# Autodesk Inventor assembly: sorting and interface V2
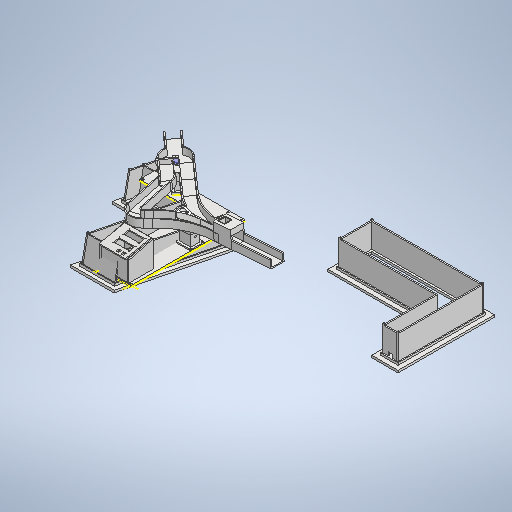
[picture p0: Inventor's stored thumbnail of the model, 512x512]
Saved by Autodesk Inventor 2025.3 (Build 293356000, 356)
## iProperties
Created: 2026-04-18
Part Number: sorting and interface V2
Document SubType Name: Assembly
Designer: kamal
Author: kamal
## Documents named in this file (30)
- C:\Users\kamal\OneDrive\Desktop\Personal\semester 4\Basics of Mechatronics\Full Assembly\sorting and interface V2.iam
- C:\Users\kamal\OneDrive\Desktop\Personal\semester 4\Basics of Mechatronics\Full Assembly\Sorting Full Mechanism.iam
- C:\Users\kamal\OneDrive\Desktop\Personal\semester 4\Basics of Mechatronics\Full Assembly\track 1832.ipt
- C:\Users\kamal\OneDrive\Desktop\Personal\semester 4\Basics of Mechatronics\Full Assembly\track z1906.ipt
- C:\Users\kamal\OneDrive\Desktop\Personal\semester 4\Basics of Mechatronics\Full Assembly\selection system 2.iam
- C:\Users\kamal\OneDrive\Desktop\Personal\semester 4\Basics of Mechatronics\Full Assembly\track z2029.ipt
- C:\Users\kamal\OneDrive\Desktop\Personal\semester 4\Basics of Mechatronics\Full Assembly\track z2053.ipt
- C:\Users\kamal\OneDrive\Desktop\Personal\semester 4\Basics of Mechatronics\Full Assembly\track z2059.ipt
- C:\Users\kamal\OneDrive\Desktop\Personal\semester 4\Basics of Mechatronics\Full Assembly\select end track.ipt
- C:\Users\kamal\OneDrive\Desktop\Personal\semester 4\Basics of Mechatronics\Full Assembly\sort support V3.ipt
- C:\Users\kamal\OneDrive\Desktop\Personal\semester 4\Basics of Mechatronics\Full Assembly\select support V3.ipt
- C:\Users\kamal\OneDrive\Desktop\Personal\semester 4\Basics of Mechatronics\Full Assembly\base zzzz.ipt
- C:\Users\kamal\OneDrive\Desktop\Personal\semester 4\Basics of Mechatronics\Full Assembly\wall inteface V1.ipt
- C:\Users\kamal\OneDrive\Desktop\Personal\semester 4\Basics of Mechatronics\Full Assembly\wall interface 2 V1.ipt
- C:\Users\kamal\OneDrive\Desktop\Personal\semester 4\Basics of Mechatronics\Full Assembly\lcd holder.ipt
- C:\Users\kamal\OneDrive\Desktop\Personal\semester 4\Basics of Mechatronics\Full Assembly\wall interface 3 V1.ipt
- C:\Users\kamal\OneDrive\Desktop\Personal\semester 4\Basics of Mechatronics\Full Assembly\base down.ipt
- C:\Users\kamal\OneDrive\Desktop\Personal\semester 4\Basics of Mechatronics\Full Assembly\wall 1 for sorting.ipt
- C:\Users\kamal\OneDrive\Desktop\Personal\semester 4\Basics of Mechatronics\Full Assembly\wall 2 for sorting.ipt
- C:\Users\kamal\OneDrive\Desktop\Personal\semester 4\Basics of Mechatronics\Full Assembly\wall 3 for sorting.ipt
- C:\Users\kamal\OneDrive\Desktop\Personal\semester 4\Basics of Mechatronics\Full Assembly\wall 4 for sorting.ipt
- C:\Users\kamal\OneDrive\Desktop\Personal\semester 4\Basics of Mechatronics\Full Assembly\wall 5 for sorting.ipt
- C:\Users\kamal\OneDrive\Desktop\Personal\semester 4\Basics of Mechatronics\Full Assembly\wall 6 for sorting.ipt
- C:\Users\kamal\OneDrive\Desktop\Personal\semester 4\Basics of Mechatronics\Full Assembly\base down_MIR.ipt
- C:\Users\kamal\OneDrive\Desktop\Personal\semester 4\Basics of Mechatronics\Full Assembly\wall 1 for sorting_MIR.ipt
- C:\Users\kamal\OneDrive\Desktop\Personal\semester 4\Basics of Mechatronics\Full Assembly\wall 2 for sorting_MIR.ipt
- C:\Users\kamal\OneDrive\Desktop\Personal\semester 4\Basics of Mechatronics\Full Assembly\wall 3 for sorting_MIR.ipt
- C:\Users\kamal\OneDrive\Desktop\Personal\semester 4\Basics of Mechatronics\Full Assembly\wall 4 for sorting_MIR.ipt
- C:\Users\kamal\OneDrive\Desktop\Personal\semester 4\Basics of Mechatronics\Full Assembly\wall 5 for sorting_MIR.ipt
- C:\Users\kamal\OneDrive\Desktop\Personal\semester 4\Basics of Mechatronics\Full Assembly\wall 6 for sorting_MIR.ipt
## Components (31 placed, 29 different names)
1. Sorting Full Mechanism:1 [sub-assembly] — Mate:12, Mate:13, Mate:14, Mate:21, Mate:22, Mate:25, Mate:26, Mate:56, Mate:57
2. track 1832:1 — Mate:12, Mate:13, Mate:14
3. track z1906:1 — Mate:21, Mate:22, Mate:52, Mate:53
4. selection system 2:1 [sub-assembly] — Mate:27, Mate:28, Mate:41, Mate:42, Mate:54, Mate:55, Mate:58, Mate:59
5. track z2029:1 — Mate:25, Mate:26, Mate:27, Mate:28
6. track z1906:3 — Mate:35, Mate:36, Mate:52, Mate:53
7. track z2053:1 — Mate:35, Mate:36
8. track z2059:1 — Mate:54, Mate:55
9. select end track:1 — Mate:41, Mate:42
10. sort support V3:1 — Mate:56, Mate:57, Mate:60, Mate:61
11. select support V3:1 — Mate:58, Mate:59
12. base zzzz:1 — Mate:60, Mate:61, Mate:62, Mate:63, Mate:64, Mate:65, Mate:68, Mate:70, Mate:98
13. wall inteface V1:1 — Mate:64, Mate:65, Mate:66, Mate:69, Mate:72
14. wall interface 2 V1:1 — Mate:62, Mate:63, Mate:67, Mate:71
15. lcd holder:1 — Mate:66
16. wall interface 3 V1:1 — Mate:69, Mate:70, Mate:71
17. wall interface 3 V1:2 — Mate:67, Mate:68, Mate:72
18. base down:1 — Mate:73, Mate:74, Mate:75, Mate:76, Mate:77, Mate:78, Mate:79, Mate:80, Mate:81, Mate:82, Mate:84
19. wall 1 for sorting:1 — Mate:73, Mate:74, Mate:85
20. wall 2 for sorting:1 — Mate:75, Mate:76
21. wall 3 for sorting:1 — Mate:77, Mate:78
22. wall 4 for sorting:1 — Mate:79, Mate:80
23. wall 5 for sorting:2 — Mate:81, Mate:82
24. wall 6 for sorting:1 — Mate:84, Mate:85
25. base down_MIR:1 — Mate:86, Mate:87, Mate:88, Mate:89, Mate:90, Mate:91, Mate:92, Mate:93, Mate:94, Mate:95, Mate:97
26. wall 1 for sorting_MIR:1 — Mate:86, Mate:87, Mate:96
27. wall 2 for sorting_MIR:1 — Mate:88, Mate:89, Mate:98
28. wall 3 for sorting_MIR:1 — Mate:90, Mate:91
29. wall 4 for sorting_MIR:1 — Mate:92, Mate:93
30. wall 5 for sorting_MIR:1 — Mate:94, Mate:95
31. wall 6 for sorting_MIR:1 — Mate:96, Mate:97
## Relationships (59: Mate 59)
- Mate:12: Sorting Full Mechanism:1 ↔ track 1832:1
- Mate:13: Sorting Full Mechanism:1 ↔ track 1832:1
- Mate:14: Sorting Full Mechanism:1 ↔ track 1832:1
- Mate:21: Sorting Full Mechanism:1 ↔ track z1906:1
- Mate:22: Sorting Full Mechanism:1 ↔ track z1906:1
- Mate:25: Sorting Full Mechanism:1 ↔ track z2029:1
- Mate:26: Sorting Full Mechanism:1 ↔ track z2029:1
- Mate:27: selection system 2:1 ↔ track z2029:1
- Mate:28: selection system 2:1 ↔ track z2029:1
- Mate:35: track z1906:3 ↔ track z2053:1
- Mate:36: track z1906:3 ↔ track z2053:1
- Mate:41: selection system 2:1 ↔ select end track:1
- Mate:42: selection system 2:1 ↔ select end track:1
- Mate:52: track z1906:1 ↔ track z1906:3
- Mate:53: track z1906:1 ↔ track z1906:3
- Mate:54: selection system 2:1 ↔ track z2059:1
- Mate:55: selection system 2:1 ↔ track z2059:1
- Mate:56: Sorting Full Mechanism:1 ↔ sort support V3:1
- Mate:57: Sorting Full Mechanism:1 ↔ sort support V3:1
- Mate:58: selection system 2:1 ↔ select support V3:1
- Mate:59 (5 mm): selection system 2:1 ↔ select support V3:1
- Mate:60: sort support V3:1 ↔ base zzzz:1
- Mate:61: sort support V3:1 ↔ base zzzz:1
- Mate:62: base zzzz:1 ↔ wall interface 2 V1:1
- Mate:63: base zzzz:1 ↔ wall interface 2 V1:1
- Mate:64: base zzzz:1 ↔ wall inteface V1:1
- Mate:65: base zzzz:1 ↔ wall inteface V1:1
- Mate:66: wall inteface V1:1 ↔ lcd holder:1
- Mate:67: wall interface 2 V1:1 ↔ wall interface 3 V1:2
- Mate:68: base zzzz:1 ↔ wall interface 3 V1:2
- Mate:69: wall inteface V1:1 ↔ wall interface 3 V1:1
- Mate:70: base zzzz:1 ↔ wall interface 3 V1:1
- Mate:71: wall interface 2 V1:1 ↔ wall interface 3 V1:1
- Mate:72: wall inteface V1:1 ↔ wall interface 3 V1:2
- Mate:73: base down:1 ↔ wall 1 for sorting:1
- Mate:74: base down:1 ↔ wall 1 for sorting:1
- Mate:75: base down:1 ↔ wall 2 for sorting:1
- Mate:76: base down:1 ↔ wall 2 for sorting:1
- Mate:77: base down:1 ↔ wall 3 for sorting:1
- Mate:78: base down:1 ↔ wall 3 for sorting:1
- Mate:79: base down:1 ↔ wall 4 for sorting:1
- Mate:80: base down:1 ↔ wall 4 for sorting:1
- Mate:81: base down:1 ↔ wall 5 for sorting:2
- Mate:82: base down:1 ↔ wall 5 for sorting:2
- Mate:84: base down:1 ↔ wall 6 for sorting:1
- Mate:85: wall 1 for sorting:1 ↔ wall 6 for sorting:1
- Mate:86: base down_MIR:1 ↔ wall 1 for sorting_MIR:1
- Mate:87: base down_MIR:1 ↔ wall 1 for sorting_MIR:1
- Mate:88: base down_MIR:1 ↔ wall 2 for sorting_MIR:1
- Mate:89: base down_MIR:1 ↔ wall 2 for sorting_MIR:1
- Mate:90: base down_MIR:1 ↔ wall 3 for sorting_MIR:1
- Mate:91: base down_MIR:1 ↔ wall 3 for sorting_MIR:1
- Mate:92: base down_MIR:1 ↔ wall 4 for sorting_MIR:1
- Mate:93: base down_MIR:1 ↔ wall 4 for sorting_MIR:1
- Mate:94: base down_MIR:1 ↔ wall 5 for sorting_MIR:1
- Mate:95: base down_MIR:1 ↔ wall 5 for sorting_MIR:1
- Mate:96: wall 1 for sorting_MIR:1 ↔ wall 6 for sorting_MIR:1
- Mate:97: base down_MIR:1 ↔ wall 6 for sorting_MIR:1
- Mate:98: base zzzz:1 ↔ wall 2 for sorting_MIR:1
